# Autodesk Inventor assembly: Base_Protesis_v6
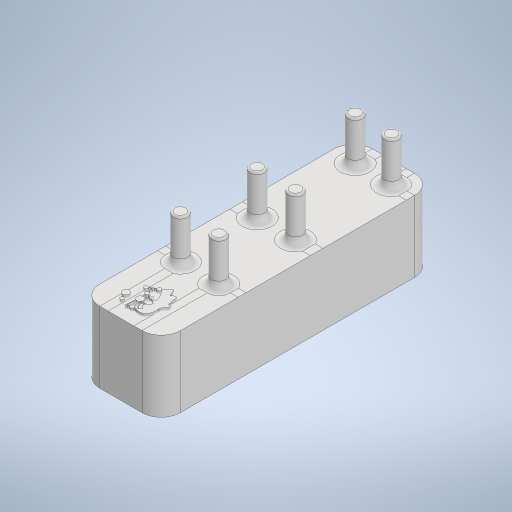
[picture p0: Inventor's stored thumbnail of the model, 512x512]
Saved by Autodesk Inventor 2024.1 (Build 281209000, 209)
## iProperties
Created: 2024-01-02
Part Number: Base_Protesis_v6
Document SubType Name: Assembly
Designer: Jonathan Zea
Author: Jonathan Zea
## Documents named in this file (3)
- Z:\Base_Protesis_v6.iam
- Z:\Base_Protesis_v4_L.ipt
- Z:\logotipo.ipt
## Components (2 placed, 2 different names)
1. Base_Protesis_v4_L:1 — Mate:1
2. logotipo:1 — Mate:1
## Relationships (1: Mate 1)
- Mate:1 (-1.3 mm): Base_Protesis_v4_L:1 ↔ logotipo:1
